# Autodesk Inventor assembly: MaleHeaderPin_1x4
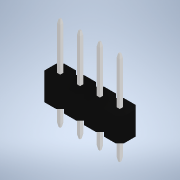
[picture p0: Inventor's stored thumbnail of the model, 180x180]
Saved by Autodesk Inventor 2021 (Build 250183000, 183)
## iProperties
Created: 2020-01-06
Part Number: MaleHeaderPin_1x4
Document SubType Name: Assembly
Designer: ermoz
Author: ermoz
## Documents named in this file (2)
- D:\Moje Wyczyny\My_Poor_Projects\Sneak100_MiniSumo\minisumo-sneak100\mechanics\PreMadeParts\MaleHeaderPin_1x4.iam
- D:\Moje Wyczyny\My_Poor_Projects\Sneak100_MiniSumo\minisumo-sneak100\mechanics\PreMadeParts\MaleHeaderPin.ipt
## Components (4 placed, 1 different names)
1. MaleHeaderPin:1 — Flush:1, Flush:8, Flush:9, Mate:1, Mate:2
2. MaleHeaderPin:2 — Flush:1, Flush:2, Flush:8, Mate:1
3. MaleHeaderPin:3 — Flush:2, Flush:3, Flush:9, Flush:10, Mate:2, Mate:3
4. MaleHeaderPin:4 — Flush:3, Flush:10, Mate:3
## Relationships (9: Flush 6, Mate 3)
- Flush:1: MaleHeaderPin:1 ↔ MaleHeaderPin:2
- Flush:2: MaleHeaderPin:2 ↔ MaleHeaderPin:3
- Flush:3: MaleHeaderPin:3 ↔ MaleHeaderPin:4
- Flush:8: MaleHeaderPin:1 ↔ MaleHeaderPin:2
- Flush:9: MaleHeaderPin:1 ↔ MaleHeaderPin:3
- Flush:10: MaleHeaderPin:3 ↔ MaleHeaderPin:4
- Mate:1: MaleHeaderPin:1 ↔ MaleHeaderPin:2
- Mate:2: MaleHeaderPin:1 ↔ MaleHeaderPin:3
- Mate:3: MaleHeaderPin:3 ↔ MaleHeaderPin:4
